# Autodesk Inventor assembly: drive
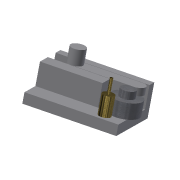
[picture p0: Inventor's stored thumbnail of the model, 180x180]
Saved by Autodesk Inventor 2022 (Build 260148000, 148)
## iProperties
Shininess: 64.0
Length Units: 11269
Angle Units: 11279
Time Units: 11290
Mass Units: 11283
Length Display Precision: 3
Angle Display Precision: 2
Created: 2001-12-31
Part Number: drive
Document SubType Name: Assembly
Designer: Administrator
Density: 0.0
Volumn: 0.0
Area: 0.0
PropertySet Name: Model Information
Control State: 0
Master: False
Checked Out: False
Author: Administrator
## Documents named in this file (5)
- C:\Autodesk Inventor 2022 Advanced Assembly Modeling Practice Files\drive.iam
- C:\Autodesk Inventor 2022 Advanced Assembly Modeling Practice Files\roll1.ipt
- C:\Autodesk Inventor 2022 Advanced Assembly Modeling Practice Files\roll2.ipt
- C:\Autodesk Inventor 2022 Advanced Assembly Modeling Practice Files\sliderarm.ipt
- C:\Autodesk Inventor 2022 Advanced Assembly Modeling Practice Files\drive_base.ipt
## Components (4 placed, 4 different names)
1. drive_base:1 — Insert:1, Insert:2, Mate:2
2. roll1:1 — Insert:1
3. roll2:1 — Mate:1, Insert:2
4. sliderarm:1 — Mate:1, Mate:2
## Relationships (4: Mate 2, Insert 2)
- Mate:1: roll2:1 ↔ sliderarm:1
- Insert:1: drive_base:1 ↔ roll1:1
- Insert:2: drive_base:1 ↔ roll2:1
- Mate:2: drive_base:1 ↔ sliderarm:1
